# Autodesk Inventor assembly: Modelado de eqilibrador
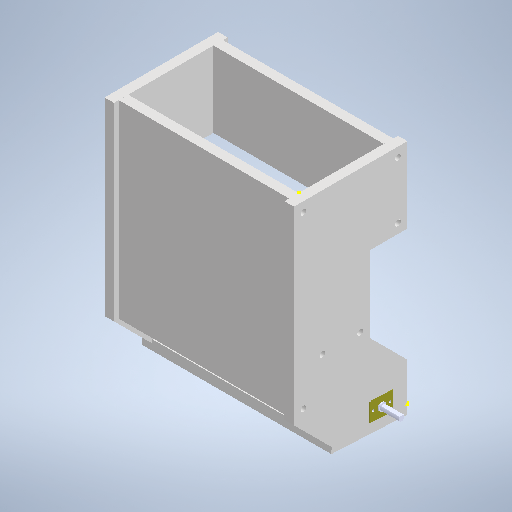
[picture p0: Inventor's stored thumbnail of the model, 512x512]
Saved by Autodesk Inventor 2025.2 (Build 292293000, 293)
## iProperties
Created: 2025-01-27
Part Number: Modelado de eqilibrador
Document SubType Name: Assembly
Designer: alex
Author: alex
## Documents named in this file (7)
- C:\Users\alex\Documents\Git\Control\Proyecto\Modelado de eqilibrador.iam
- C:\Users\alex\Documents\Git\Control\Proyecto\Base.ipt
- C:\Users\alex\Documents\Git\Control\Proyecto\Atras.ipt
- C:\Users\alex\Documents\Git\Control\Proyecto\Lateral.ipt
- C:\Users\alex\Documents\Git\Control\Proyecto\Interno.ipt
- C:\Users\alex\Documents\Git\Control\Proyecto\Frontal.ipt
- C:\Users\alex\Documents\Git\Control\Proyecto\N20 Motor.ipt
## Components (8 placed, 6 different names)
1. Lateral:1 — Insertar:1, Coincidencia:1, Insertar:3
2. Atras:1 — Insertar:1, Insertar:2
3. Lateral:2 — Insertar:2, Coincidencia:2, Coincidencia:3, Insertar:4
4. Base:1 — Coincidencia:1, Coincidencia:2, Insertar:5, Insertar:6, Insertar:7, Insertar:8
5. Frontal:1 — Coincidencia:3, Insertar:3
6. Interno:1 — Insertar:4
7. N20 Motor:1 — Insertar:5, Insertar:6
8. N20 Motor:2 — Insertar:7, Insertar:8
## Relationships (11: Insert 8, Mate 3)
- Insertar:1: Lateral:1 ↔ Atras:1
- Insertar:2: Atras:1 ↔ Lateral:2
- Coincidencia:1 [Mate]: Lateral:1 ↔ Base:1
- Coincidencia:2 [Mate]: Lateral:2 ↔ Base:1
- Coincidencia:3 [Mate]: Lateral:2 ↔ Frontal:1
- Insertar:3: Lateral:1 ↔ Frontal:1
- Insertar:4: Lateral:2 ↔ Interno:1
- Insertar:5: Base:1 ↔ N20 Motor:1
- Insertar:6: Base:1 ↔ N20 Motor:1
- Insertar:7: Base:1 ↔ N20 Motor:2
- Insertar:8: Base:1 ↔ N20 Motor:2
